# Autodesk Inventor assembly: Assembly_NoStepper
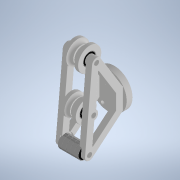
[picture p0: Inventor's stored thumbnail of the model, 180x180]
Saved by Autodesk Inventor 2021 (Build 250183000, 183)
## iProperties
Created: 2021-07-14
Part Number: Assembly_NoStepper
Document SubType Name: Assembly
Designer: zmac845
Author: zmac845
## Documents named in this file (5)
- \\files.auckland.ac.nz\myhome\Documents\Year 4\MECHENG 700\Test 8 July\Assembly_NoStepper.iam
- \\files.auckland.ac.nz\myhome\Documents\Year 4\MECHENG 700\Test 8 July\Frame.ipt
- \\files.auckland.ac.nz\myhome\Documents\Year 4\MECHENG 700\Hand Extruder\Bearing.ipt
- \\files.auckland.ac.nz\myhome\Documents\Year 4\MECHENG 700\Test 8 July\LeadWheelHalf.ipt
- \\files.auckland.ac.nz\myhome\Documents\Year 4\MECHENG 700\Test 8 July\DriveWheelHalf.ipt
## Components (14 placed, 4 different names)
1. Frame:1 — Rotational:1, Rotational:2, Rotational:3, Rotational:4, Rotational:9
2. Bearing:1 — Rotational:1, Rotational:12
3. Bearing:2 — Rotational:2, Rotational:11
4. Bearing:3 — Rotational:5, Rotational:6
5. Bearing:4 — Rotational:6, Rotational:7
6. Bearing:5 — Rotational:7, Rotational:8
7. Bearing:6 — Rotational:3, Rotational:14
8. Bearing:7 — Rotational:4, Rotational:5
9. Bearing:8 — Rotational:8
10. Bearing:9 — Rotational:9, Rotational:13
11. LeadWheelHalf:1 — Rotational:12
12. LeadWheelHalf:2 — Rotational:11
13. DriveWheelHalf:1 — Rotational:13
14. DriveWheelHalf:2 — Rotational:14
## Relationships (13: RevoluteJoint 13)
- Rotational:1 [RevoluteJoint]: Frame:1 ↔ Bearing:1
- Rotational:2 [RevoluteJoint]: Frame:1 ↔ Bearing:2
- Rotational:3 [RevoluteJoint]: Frame:1 ↔ Bearing:6
- Rotational:4 [RevoluteJoint]: Frame:1 ↔ Bearing:7
- Rotational:5 [RevoluteJoint]: Bearing:3 ↔ Bearing:7
- Rotational:6 [RevoluteJoint]: Bearing:3 ↔ Bearing:4
- Rotational:7 [RevoluteJoint]: Bearing:4 ↔ Bearing:5
- Rotational:8 [RevoluteJoint]: Bearing:5 ↔ Bearing:8
- Rotational:9 [RevoluteJoint]: Frame:1 ↔ Bearing:9
- Rotational:11 [RevoluteJoint]: Bearing:2 ↔ LeadWheelHalf:2
- Rotational:12 [RevoluteJoint]: Bearing:1 ↔ LeadWheelHalf:1
- Rotational:13 [RevoluteJoint]: Bearing:9 ↔ DriveWheelHalf:1
- Rotational:14 [RevoluteJoint]: Bearing:6 ↔ DriveWheelHalf:2
